# Autodesk Inventor assembly: Assembly1TankDrive
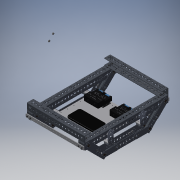
[picture p0: Inventor's stored thumbnail of the model, 180x180]
Saved by Autodesk Inventor 2016 (Build 200138000, 138)
## iProperties
Created: 2015-09-29
Part Number: Assembly1TankDrive
Document SubType Name: Assembly
Designer: phiro
Author: phiro
## Documents named in this file (15)
- C:\Users\phiro\Documents\GitHub\phi_robotics\3d-models\FTC_Tetrix_KOP_Block_Party\Troy designs\Assembly1TankDrive.iam
- C:\Users\phiro\Documents\GitHub\phi_robotics\3d-models\FTC_Tetrix_KOP_Block_Party\Tetrix_Kit_FTC\Autodesk Inventor Files\tetrix_c_channel-5.ipt
- C:\Users\phiro\Documents\GitHub\phi_robotics\3d-models\FTC_Tetrix_KOP_Block_Party\Tetrix_Kit_FTC\Autodesk Inventor Files\tetrix_739061_2012.ipt
- C:\Users\phiro\Documents\GitHub\phi_robotics\3d-models\FTC_Tetrix_KOP_Block_Party\Tetrix_Kit_FTC\Autodesk Inventor Files\tetrix_c_channel-2.ipt
- C:\Users\phiro\Documents\GitHub\phi_robotics\3d-models\FTC_Tetrix_KOP_Block_Party\Tetrix_Kit_FTC\Autodesk Inventor Files\tetrix_c_channel-3.ipt
- C:\Users\phiro\Documents\GitHub\phi_robotics\3d-models\FTC_Tetrix_KOP_Block_Party\Tetrix_Kit_FTC\Autodesk Inventor Files\tetrix_c_channel-4.ipt
- C:\Users\phiro\Documents\GitHub\phi_robotics\3d-models\FTC_Tetrix_KOP_Block_Party\Tetrix_Kit_FTC\Autodesk Inventor Files\tetrix_Lbracket-round.ipt
- C:\Users\phiro\Documents\GitHub\phi_robotics\3d-models\FTC_Tetrix_KOP_Block_Party\Tetrix_Kit_FTC\Autodesk Inventor Files\tetrix_flat_bar-288 MM.ipt
- C:\Users\phiro\Documents\GitHub\phi_robotics\3d-models\FTC_Tetrix_KOP_Block_Party\Tetrix_Kit_FTC\Autodesk Inventor Files\tetrix_screw-short.ipt
- C:\Users\phiro\Documents\GitHub\phi_robotics\3d-models\FTC_Tetrix_KOP_Block_Party\Tetrix_Kit_FTC\Autodesk Inventor Files\tetrix_lock_nut.ipt
- C:\Users\phiro\Documents\GitHub\phi_robotics\3d-models\FTC_Tetrix_KOP_Block_Party\Tetrix_Kit_FTC\Autodesk Inventor Files\tetrix_bushing.ipt
- C:\Users\phiro\Documents\GitHub\phi_robotics\3d-models\FTC_Tetrix_KOP_Block_Party\Tim Bloot Designs\MCPlate2.ipt
- C:\Users\phiro\Documents\GitHub\phi_robotics\3d-models\FTC_Tetrix_KOP_Block_Party\Tetrix_Kit_FTC\Autodesk Inventor Files\tetrix_739274_2013.ipt
- C:\Users\phiro\Documents\GitHub\phi_robotics\3d-models\FTC_Tetrix_KOP_Block_Party\Tim Bloot Designs\Andoid Phone.ipt
- C:\Users\phiro\Documents\GitHub\phi_robotics\3d-models\FTC_Tetrix_KOP_Block_Party\Tetrix_Kit_FTC\Autodesk Inventor Files\tetrix_motor_controller.ipt
## Components (222 placed, 14 different names)
1. tetrix_739061_2012:1 — Rigid:2, Rigid:58, Rigid:162, Rigid:163, Rigid:164, Rigid:165
2. tetrix_739061_2012:2 — Rigid:1, Rigid:3, Rigid:59, Rigid:166, Rigid:167, Rigid:168, Rigid:169
3. tetrix_c_channel-2:1 — Rigid:3, Rigid:6, Rigid:8, Rigid:196, Rigid:197, Rigid:198, Rigid:199, Rigid:212, Rigid:213, Rigid:214, Rigid:215
4. tetrix_739061_2012:3 — Rigid:4, Rigid:61, Rigid:178, Rigid:179, Rigid:180, Rigid:181
5. tetrix_739061_2012:4 — Rigid:5, Rotational:1, Rigid:60, Rigid:150, Rigid:151, Rigid:152, Rigid:153
6. tetrix_c_channel-2:2 — Rotational:1, Rigid:7, Rigid:9, Rigid:204, Rigid:205, Rigid:206, Rigid:207, Rigid:220, Rigid:221, Rigid:222, Rigid:223
7. tetrix_c_channel-3:1 — Rigid:10, Rigid:202, Rigid:203, Rigid:218, Rigid:219
8. tetrix_739061_2012:5 — Rigid:7, Rigid:10, Rigid:69, Rigid:174, Rigid:175, Rigid:176, Rigid:177
9. tetrix_739061_2012:6 — Rigid:9, Rigid:65, Rigid:154, Rigid:155, Rigid:156, Rigid:157
10. tetrix_739061_2012:7 — Rigid:8, Rigid:64, Rigid:158, Rigid:159, Rigid:160, Rigid:161
11. tetrix_739061_2012:8 — Rigid:6, Rigid:68, Rigid:170, Rigid:171, Rigid:172, Rigid:173
12. tetrix_c_channel-5:2 — Rigid:22, Rigid:23, Rigid:27, Rigid:29, Rigid:102, Rigid:103, Rigid:116, Rigid:117, Rigid:134, Rigid:135, Rigid:148, Rigid:149, Rigid:182, Rigid:183
13. tetrix_739061_2012:9 — Rigid:55, Rigid:86, Rigid:87, Rigid:88, Rigid:89
14. tetrix_739061_2012:10 — Rigid:54, Rigid:118, Rigid:119, Rigid:120, Rigid:121
15. tetrix_c_channel-2:3 — Rigid:104, Rigid:105, Rigid:106, Rigid:107, Rigid:136, Rigid:137, Rigid:138, Rigid:139
16. tetrix_739061_2012:11 — Rigid:56, Rigid:130, Rigid:131, Rigid:132, Rigid:133
17. tetrix_739061_2012:12 — Rotational:2, Rigid:57, Rigid:92, Rigid:93, Rigid:94, Rigid:95
18. tetrix_739061_2012:15 — Rigid:67, Rigid:90, Rigid:91, Rigid:100, Rigid:101
19. tetrix_739061_2012:16 — Rigid:62, Rigid:122, Rigid:123, Rigid:124, Rigid:125
20. tetrix_c_channel-4:1 — Rigid:21, Rigid:22, Rigid:70, Rigid:71, Rigid:74, Rigid:75
21. tetrix_c_channel-4:2 — Rigid:23, Rigid:72, Rigid:73, Rigid:76, Rigid:77
22. tetrix_c_channel-2:4 — Rotational:2, Rigid:24, Rigid:25, Rigid:112, Rigid:113, Rigid:114, Rigid:115, Rigid:144, Rigid:145, Rigid:146, Rigid:147
23. tetrix_739061_2012:17 — Rigid:24, Rigid:26, Rigid:63, Rigid:126, Rigid:127, Rigid:128, Rigid:129
24. tetrix_739061_2012:18 — Rigid:25, Rigid:66, Rigid:96, Rigid:97, Rigid:98, Rigid:99
25. tetrix_c_channel-3:2 — Rigid:26, Rigid:110, Rigid:111, Rigid:142, Rigid:143
26. tetrix_Lbracket-round:1 — Rigid:27, Rigid:31, Rigid:34, Rigid:36, Rigid:78, Rigid:79
27. tetrix_Lbracket-round:2 — Rigid:28, Rigid:39, Rigid:40, Rigid:82, Rigid:83
28. tetrix_Lbracket-round:3 — Rigid:29, Rigid:43, Rigid:44, Rigid:80, Rigid:81
29. tetrix_Lbracket-round:4 — Rigid:30, Rigid:32, Rigid:47, Rigid:48, Rigid:84, Rigid:85
30. tetrix_flat_bar-288 MM:1 — Rigid:31, Rigid:33, Rigid:35, Rigid:37, Rigid:38
31. tetrix_flat_bar-288 MM:2 — Rigid:32, Rigid:41, Rigid:42, Rigid:45, Rigid:46
32. tetrix_screw-short:1 — Rigid:33
33. tetrix_lock_nut:1 — Rigid:34
34. tetrix_screw-short:2 — Rigid:35
35. tetrix_screw-short:3 — Rigid:38
36. tetrix_screw-short:4 — Rigid:37
37. tetrix_screw-short:5 — Rigid:41
38. tetrix_screw-short:6 — Rigid:42
39. tetrix_screw-short:7 — Rigid:46
40. tetrix_screw-short:8 — Rigid:45
41. tetrix_lock_nut:2 — Rigid:36
42. tetrix_lock_nut:3 — Rigid:39
43. tetrix_lock_nut:4 — Rigid:40
44. tetrix_lock_nut:5 — Rigid:43
45. tetrix_lock_nut:6 — Rigid:44
46. tetrix_lock_nut:7 — Rigid:47
47. tetrix_lock_nut:8 — Rigid:48
48. tetrix_bushing:1 — Rigid:54
49. tetrix_bushing:2 — Rigid:56
50. tetrix_bushing:3 — Rigid:55
51. tetrix_bushing:4 — Rigid:57
52. tetrix_bushing:5 — Rigid:58
53. tetrix_bushing:6 — Rigid:60
54. tetrix_bushing:8 — Rigid:61
55. tetrix_bushing:9 — Rigid:59
56. tetrix_bushing:10 — Rigid:66
57. tetrix_bushing:11 — Rigid:67
58. tetrix_bushing:12 — Rigid:64
59. tetrix_bushing:13 — Rigid:65
60. tetrix_bushing:14 — Rigid:63
61. tetrix_bushing:15 — Rigid:62
62. tetrix_bushing:16 — Rigid:68
63. tetrix_bushing:17 — Rigid:69
64. tetrix_screw-short:9 — Rigid:71
65. tetrix_screw-short:10 — Rigid:70
66. tetrix_screw-short:11 — Rigid:72
67. tetrix_screw-short:12 — Rigid:73
68. tetrix_screw-short:13 — Rigid:77
69. tetrix_screw-short:14 — Rigid:76
70. tetrix_screw-short:15 — Rigid:75
71. tetrix_screw-short:16 — Rigid:74
72. tetrix_lock_nut:9 — Rigid:78
73. tetrix_lock_nut:10 — Rigid:79
74. tetrix_lock_nut:11 — Rigid:80
75. tetrix_lock_nut:12 — Rigid:81
76. tetrix_lock_nut:13 — Rigid:84
77. tetrix_lock_nut:14 — Rigid:85
78. tetrix_lock_nut:15 — Rigid:82
79. tetrix_lock_nut:16 — Rigid:83
80. tetrix_screw-short:17 — Rigid:87
81. tetrix_screw-short:18 — Rigid:86
82. tetrix_screw-short:19 — Rigid:91
83. tetrix_screw-short:20 — Rigid:89
84. tetrix_screw-short:21 — Rigid:90
85. tetrix_screw-short:22 — Rigid:88
86. tetrix_screw-short:23 — Rigid:95
87. tetrix_screw-short:24 — Rigid:94
88. tetrix_screw-short:25 — Rigid:97
89. tetrix_screw-short:26 — Rigid:96
90. tetrix_screw-short:27 — Rigid:93
91. tetrix_screw-short:28 — Rigid:92
92. tetrix_screw-short:29 — Rigid:99
93. tetrix_screw-short:30 — Rigid:98
94. tetrix_screw-short:31 — Rigid:100, Rigid:108
95. tetrix_screw-short:32 — Rigid:101, Rigid:109
96. tetrix_lock_nut:17 — Rigid:102
97. tetrix_lock_nut:18 — Rigid:103
98. tetrix_lock_nut:19 — Rigid:104
99. tetrix_lock_nut:20 — Rigid:105
100. tetrix_lock_nut:21 — Rigid:106
101. tetrix_lock_nut:22 — Rigid:107
102. tetrix_lock_nut:23 — Rigid:108
103. tetrix_lock_nut:24 — Rigid:109
104. tetrix_lock_nut:25 — Rigid:110
105. tetrix_lock_nut:26 — Rigid:111
106. tetrix_lock_nut:27 — Rigid:112
107. tetrix_lock_nut:28 — Rigid:113
108. tetrix_lock_nut:29 — Rigid:114
109. tetrix_lock_nut:30 — Rigid:115
110. tetrix_lock_nut:31 — Rigid:116
111. tetrix_lock_nut:32 — Rigid:117
112. tetrix_screw-short:33 — Rigid:119
113. tetrix_screw-short:34 — Rigid:118
114. tetrix_screw-short:35 — Rigid:120
115. tetrix_screw-short:36 — Rigid:121
116. tetrix_screw-short:37 — Rigid:122
117. tetrix_screw-short:38 — Rigid:123
118. tetrix_screw-short:39 — Rigid:124, Rigid:140
119. tetrix_screw-short:40 — Rigid:125, Rigid:141
120. tetrix_screw-short:41 — Rigid:126
121. tetrix_screw-short:42 — Rigid:127
122. tetrix_screw-short:43 — Rigid:128
123. tetrix_screw-short:44 — Rigid:129
124. tetrix_screw-short:45 — Rigid:130
125. tetrix_screw-short:46 — Rigid:131
126. tetrix_screw-short:47 — Rigid:132
127. tetrix_screw-short:48 — Rigid:133
128. tetrix_lock_nut:33 — Rigid:134
129. tetrix_lock_nut:34 — Rigid:135
130. tetrix_lock_nut:35 — Rigid:136
131. tetrix_lock_nut:36 — Rigid:137
132. tetrix_lock_nut:37 — Rigid:138
133. tetrix_lock_nut:38 — Rigid:139
134. tetrix_lock_nut:39 — Rigid:140
135. tetrix_lock_nut:40 — Rigid:141
136. tetrix_lock_nut:41 — Rigid:142
137. tetrix_lock_nut:42 — Rigid:143
138. tetrix_lock_nut:43 — Rigid:144
139. tetrix_lock_nut:44 — Rigid:145
140. tetrix_lock_nut:45 — Rigid:146
141. tetrix_lock_nut:46 — Rigid:147
142. tetrix_lock_nut:47 — Rigid:148
143. tetrix_lock_nut:48 — Rigid:149
144. tetrix_screw-short:49 — Rigid:150
145. tetrix_screw-short:50 — Rigid:151
146. tetrix_screw-short:51 — Rigid:152
147. tetrix_screw-short:52 — Rigid:153
148. tetrix_screw-short:53 — Rigid:154
149. tetrix_screw-short:54 — Rigid:155
150. tetrix_screw-short:55 — Rigid:156
151. tetrix_screw-short:56 — Rigid:157
152. tetrix_screw-short:57 — Rigid:158, Rigid:217
153. tetrix_screw-short:58 — Rigid:159, Rigid:216
154. tetrix_screw-short:59 — Rigid:160
155. tetrix_screw-short:60 — Rigid:161
156. tetrix_screw-short:61 — Rigid:162
157. tetrix_screw-short:62 — Rigid:163
158. tetrix_screw-short:63 — Rigid:164
159. tetrix_screw-short:64 — Rigid:165
160. tetrix_screw-short:65 — Rigid:181
161. tetrix_screw-short:66 — Rigid:180
162. tetrix_screw-short:67 — Rigid:179
163. tetrix_screw-short:68 — Rigid:178
164. tetrix_screw-short:69 — Rigid:177
165. tetrix_screw-short:70 — Rigid:176
166. tetrix_screw-short:71 — Rigid:175
167. tetrix_screw-short:72 — Rigid:174
168. tetrix_screw-short:73 — Rigid:173, Rigid:201
169. tetrix_screw-short:74 — Rigid:172, Rigid:200
170. tetrix_screw-short:75 — Rigid:171
171. tetrix_screw-short:76 — Rigid:170
172. tetrix_screw-short:77 — Rigid:169
173. tetrix_screw-short:78 — Rigid:168
174. tetrix_screw-short:79 — Rigid:167
175. tetrix_screw-short:80 — Rigid:166
176. MCPlate2:1 — Rigid:192, Mate:1, Rigid:193, Rotational:3
177. tetrix_flat_bar-288 MM:3 — Rigid:190
178. tetrix_flat_bar-288 MM:4 — Rigid:191, Rigid:192
179. tetrix_739274_2013:1 — Rigid:183, Rigid:187
180. tetrix_739274_2013:2 — Rigid:182, Rigid:186
181. tetrix_739274_2013:3 — Rigid:185, Rigid:189
182. tetrix_739274_2013:4 — Rigid:184, Rigid:188
183. tetrix_Lbracket-round:5 — Rigid:188, Rigid:190
184. tetrix_Lbracket-round:6 — Rigid:189
185. tetrix_Lbracket-round:7 — Rigid:186
186. tetrix_Lbracket-round:8 — Rigid:187, Rigid:191
187. Andoid Phone:1 — Mate:1
188. tetrix_motor_controller:1 — Rigid:193
189. tetrix_motor_controller:2 — Rotational:3
190. tetrix_lock_nut:49 — Rigid:210
191. tetrix_lock_nut:50 — Rigid:211
192. tetrix_lock_nut:51 — Rigid:212
193. tetrix_lock_nut:52 — Rigid:213
194. tetrix_lock_nut:53 — Rigid:214
195. tetrix_lock_nut:54 — Rigid:215
196. tetrix_lock_nut:55 — Rigid:216
197. tetrix_lock_nut:56 — Rigid:217
198. tetrix_lock_nut:57 — Rigid:218
199. tetrix_lock_nut:58 — Rigid:219
200. tetrix_lock_nut:59 — Rigid:220
201. tetrix_lock_nut:60 — Rigid:221
202. tetrix_lock_nut:61 — Rigid:222
203. tetrix_lock_nut:62 — Rigid:223
204. tetrix_lock_nut:63
205. tetrix_lock_nut:64
206. tetrix_lock_nut:65 — Rigid:194
207. tetrix_lock_nut:66 — Rigid:195
208. tetrix_lock_nut:67 — Rigid:196
209. tetrix_lock_nut:68 — Rigid:197
210. tetrix_lock_nut:69 — Rigid:198
211. tetrix_lock_nut:70 — Rigid:200
212. tetrix_lock_nut:71 — Rigid:199
213. tetrix_lock_nut:72 — Rigid:201
214. tetrix_lock_nut:73 — Rigid:202
215. tetrix_lock_nut:74 — Rigid:203
216. tetrix_lock_nut:75 — Rigid:204
217. tetrix_lock_nut:76 — Rigid:205
218. tetrix_lock_nut:77 — Rigid:206
219. tetrix_lock_nut:78 — Rigid:207
220. tetrix_lock_nut:79 — Rigid:208
221. tetrix_lock_nut:80 — Rigid:209
222. tetrix_c_channel-5:1 — Rigid:1, Rigid:2, Rigid:4, Rigid:5, Rigid:21, Rigid:28, Rigid:30, Rigid:184, Rigid:185, Rigid:194, Rigid:195, Rigid:208, Rigid:209, Rigid:210, Rigid:211
## Relationships (219: WeldJoint 215, RevoluteJoint 3, Mate 1)
- Rigid:1 [WeldJoint]: tetrix_739061_2012:2 ↔ tetrix_c_channel-5:1
- Rigid:2 [WeldJoint]: tetrix_739061_2012:1 ↔ tetrix_c_channel-5:1
- Rigid:3 [WeldJoint]: tetrix_739061_2012:2 ↔ tetrix_c_channel-2:1
- Rigid:4 [WeldJoint]: tetrix_739061_2012:3 ↔ tetrix_c_channel-5:1
- Rigid:5 [WeldJoint]: tetrix_739061_2012:4 ↔ tetrix_c_channel-5:1
- Rotational:1 [RevoluteJoint]: tetrix_739061_2012:4 ↔ tetrix_c_channel-2:2
- Rigid:6 [WeldJoint]: tetrix_c_channel-2:1 ↔ tetrix_739061_2012:8
- Rigid:7 [WeldJoint]: tetrix_c_channel-2:2 ↔ tetrix_739061_2012:5
- Rigid:8 [WeldJoint]: tetrix_c_channel-2:1 ↔ tetrix_739061_2012:7
- Rigid:9 [WeldJoint]: tetrix_c_channel-2:2 ↔ tetrix_739061_2012:6
- Rigid:10 [WeldJoint]: tetrix_c_channel-3:1 ↔ tetrix_739061_2012:5
- [WeldJoint]: tetrix_c_channel-5:2 ↔ tetrix_739061_2012:10
- [WeldJoint]: tetrix_c_channel-5:2 ↔ tetrix_739061_2012:9
- [WeldJoint]: tetrix_739061_2012:10 ↔ tetrix_c_channel-2:3
- [WeldJoint]: tetrix_c_channel-5:2 ↔ tetrix_739061_2012:11
- [WeldJoint]: tetrix_c_channel-5:2 ↔ tetrix_739061_2012:12
- [WeldJoint]: tetrix_c_channel-2:3 ↔ tetrix_739061_2012:16
- [WeldJoint]: tetrix_c_channel-2:3 ↔ tetrix_739061_2012:15
- Rigid:21 [WeldJoint]: tetrix_c_channel-4:1 ↔ tetrix_c_channel-5:1
- Rigid:22 [WeldJoint]: tetrix_c_channel-5:2 ↔ tetrix_c_channel-4:1
- Rigid:23 [WeldJoint]: tetrix_c_channel-5:2 ↔ tetrix_c_channel-4:2
- Rotational:2 [RevoluteJoint]: tetrix_739061_2012:12 ↔ tetrix_c_channel-2:4
- Rigid:24 [WeldJoint]: tetrix_c_channel-2:4 ↔ tetrix_739061_2012:17
- Rigid:25 [WeldJoint]: tetrix_c_channel-2:4 ↔ tetrix_739061_2012:18
- Rigid:26 [WeldJoint]: tetrix_739061_2012:17 ↔ tetrix_c_channel-3:2
- Rigid:27 [WeldJoint]: tetrix_c_channel-5:2 ↔ tetrix_Lbracket-round:1
- Rigid:28 [WeldJoint]: tetrix_Lbracket-round:2 ↔ tetrix_c_channel-5:1
- Rigid:29 [WeldJoint]: tetrix_c_channel-5:2 ↔ tetrix_Lbracket-round:3
- Rigid:30 [WeldJoint]: tetrix_Lbracket-round:4 ↔ tetrix_c_channel-5:1
- Rigid:31 [WeldJoint]: tetrix_Lbracket-round:1 ↔ tetrix_flat_bar-288 MM:1
- Rigid:32 [WeldJoint]: tetrix_Lbracket-round:4 ↔ tetrix_flat_bar-288 MM:2
- Rigid:33 [WeldJoint]: tetrix_flat_bar-288 MM:1 ↔ tetrix_screw-short:1
- Rigid:34 [WeldJoint]: tetrix_Lbracket-round:1 ↔ tetrix_lock_nut:1
- Rigid:35 [WeldJoint]: tetrix_flat_bar-288 MM:1 ↔ tetrix_screw-short:2
- Rigid:36 [WeldJoint]: tetrix_Lbracket-round:1 ↔ tetrix_lock_nut:2
- Rigid:37 [WeldJoint]: tetrix_flat_bar-288 MM:1 ↔ tetrix_screw-short:4
- Rigid:38 [WeldJoint]: tetrix_flat_bar-288 MM:1 ↔ tetrix_screw-short:3
- Rigid:39 [WeldJoint]: tetrix_Lbracket-round:2 ↔ tetrix_lock_nut:3
- Rigid:40 [WeldJoint]: tetrix_Lbracket-round:2 ↔ tetrix_lock_nut:4
- Rigid:41 [WeldJoint]: tetrix_flat_bar-288 MM:2 ↔ tetrix_screw-short:5
- Rigid:42 [WeldJoint]: tetrix_flat_bar-288 MM:2 ↔ tetrix_screw-short:6
- Rigid:43 [WeldJoint]: tetrix_Lbracket-round:3 ↔ tetrix_lock_nut:5
- Rigid:44 [WeldJoint]: tetrix_Lbracket-round:3 ↔ tetrix_lock_nut:6
- Rigid:45 [WeldJoint]: tetrix_flat_bar-288 MM:2 ↔ tetrix_screw-short:8
- Rigid:46 [WeldJoint]: tetrix_flat_bar-288 MM:2 ↔ tetrix_screw-short:7
- Rigid:47 [WeldJoint]: tetrix_Lbracket-round:4 ↔ tetrix_lock_nut:7
- Rigid:48 [WeldJoint]: tetrix_Lbracket-round:4 ↔ tetrix_lock_nut:8
- Rigid:54 [WeldJoint]: tetrix_739061_2012:10 ↔ tetrix_bushing:1
- Rigid:55 [WeldJoint]: tetrix_739061_2012:9 ↔ tetrix_bushing:3
- Rigid:56 [WeldJoint]: tetrix_739061_2012:11 ↔ tetrix_bushing:2
- Rigid:57 [WeldJoint]: tetrix_739061_2012:12 ↔ tetrix_bushing:4
- Rigid:58 [WeldJoint]: tetrix_739061_2012:1 ↔ tetrix_bushing:5
- Rigid:59 [WeldJoint]: tetrix_739061_2012:2 ↔ tetrix_bushing:9
- Rigid:60 [WeldJoint]: tetrix_739061_2012:4 ↔ tetrix_bushing:6
- Rigid:61 [WeldJoint]: tetrix_739061_2012:3 ↔ tetrix_bushing:8
- Rigid:62 [WeldJoint]: tetrix_739061_2012:16 ↔ tetrix_bushing:15
- Rigid:63 [WeldJoint]: tetrix_739061_2012:17 ↔ tetrix_bushing:14
- Rigid:64 [WeldJoint]: tetrix_739061_2012:7 ↔ tetrix_bushing:12
- Rigid:65 [WeldJoint]: tetrix_739061_2012:6 ↔ tetrix_bushing:13
- Rigid:66 [WeldJoint]: tetrix_739061_2012:18 ↔ tetrix_bushing:10
- Rigid:67 [WeldJoint]: tetrix_739061_2012:15 ↔ tetrix_bushing:11
- Rigid:68 [WeldJoint]: tetrix_739061_2012:8 ↔ tetrix_bushing:16
- Rigid:69 [WeldJoint]: tetrix_739061_2012:5 ↔ tetrix_bushing:17
- Rigid:70 [WeldJoint]: tetrix_c_channel-4:1 ↔ tetrix_screw-short:10
- Rigid:71 [WeldJoint]: tetrix_c_channel-4:1 ↔ tetrix_screw-short:9
- Rigid:72 [WeldJoint]: tetrix_c_channel-4:2 ↔ tetrix_screw-short:11
- Rigid:73 [WeldJoint]: tetrix_c_channel-4:2 ↔ tetrix_screw-short:12
- Rigid:74 [WeldJoint]: tetrix_c_channel-4:1 ↔ tetrix_screw-short:16
- Rigid:75 [WeldJoint]: tetrix_c_channel-4:1 ↔ tetrix_screw-short:15
- Rigid:76 [WeldJoint]: tetrix_c_channel-4:2 ↔ tetrix_screw-short:14
- Rigid:77 [WeldJoint]: tetrix_c_channel-4:2 ↔ tetrix_screw-short:13
- Rigid:78 [WeldJoint]: tetrix_Lbracket-round:1 ↔ tetrix_lock_nut:9
- Rigid:79 [WeldJoint]: tetrix_Lbracket-round:1 ↔ tetrix_lock_nut:10
- Rigid:80 [WeldJoint]: tetrix_Lbracket-round:3 ↔ tetrix_lock_nut:11
- Rigid:81 [WeldJoint]: tetrix_Lbracket-round:3 ↔ tetrix_lock_nut:12
- Rigid:82 [WeldJoint]: tetrix_Lbracket-round:2 ↔ tetrix_lock_nut:15
- Rigid:83 [WeldJoint]: tetrix_Lbracket-round:2 ↔ tetrix_lock_nut:16
- Rigid:84 [WeldJoint]: tetrix_Lbracket-round:4 ↔ tetrix_lock_nut:13
- Rigid:85 [WeldJoint]: tetrix_Lbracket-round:4 ↔ tetrix_lock_nut:14
- Rigid:86 [WeldJoint]: tetrix_739061_2012:9 ↔ tetrix_screw-short:18
- Rigid:87 [WeldJoint]: tetrix_739061_2012:9 ↔ tetrix_screw-short:17
- Rigid:88 [WeldJoint]: tetrix_739061_2012:9 ↔ tetrix_screw-short:22
- Rigid:89 [WeldJoint]: tetrix_739061_2012:9 ↔ tetrix_screw-short:20
- Rigid:90 [WeldJoint]: tetrix_739061_2012:15 ↔ tetrix_screw-short:21
- Rigid:91 [WeldJoint]: tetrix_739061_2012:15 ↔ tetrix_screw-short:19
- Rigid:92 [WeldJoint]: tetrix_739061_2012:12 ↔ tetrix_screw-short:28
- Rigid:93 [WeldJoint]: tetrix_739061_2012:12 ↔ tetrix_screw-short:27
- Rigid:94 [WeldJoint]: tetrix_739061_2012:12 ↔ tetrix_screw-short:24
- Rigid:95 [WeldJoint]: tetrix_739061_2012:12 ↔ tetrix_screw-short:23
- Rigid:96 [WeldJoint]: tetrix_739061_2012:18 ↔ tetrix_screw-short:26
- Rigid:97 [WeldJoint]: tetrix_739061_2012:18 ↔ tetrix_screw-short:25
- Rigid:98 [WeldJoint]: tetrix_739061_2012:18 ↔ tetrix_screw-short:30
- Rigid:99 [WeldJoint]: tetrix_739061_2012:18 ↔ tetrix_screw-short:29
- Rigid:100 [WeldJoint]: tetrix_739061_2012:15 ↔ tetrix_screw-short:31
- Rigid:101 [WeldJoint]: tetrix_739061_2012:15 ↔ tetrix_screw-short:32
- Rigid:102 [WeldJoint]: tetrix_c_channel-5:2 ↔ tetrix_lock_nut:17
- Rigid:103 [WeldJoint]: tetrix_c_channel-5:2 ↔ tetrix_lock_nut:18
- Rigid:104 [WeldJoint]: tetrix_c_channel-2:3 ↔ tetrix_lock_nut:19
- Rigid:105 [WeldJoint]: tetrix_c_channel-2:3 ↔ tetrix_lock_nut:20
- Rigid:106 [WeldJoint]: tetrix_c_channel-2:3 ↔ tetrix_lock_nut:21
- Rigid:107 [WeldJoint]: tetrix_c_channel-2:3 ↔ tetrix_lock_nut:22
- Rigid:108 [WeldJoint] (3 mm): tetrix_screw-short:31 ↔ tetrix_lock_nut:23
- Rigid:109 [WeldJoint] (3 mm): tetrix_screw-short:32 ↔ tetrix_lock_nut:24
- Rigid:110 [WeldJoint]: tetrix_c_channel-3:2 ↔ tetrix_lock_nut:25
- Rigid:111 [WeldJoint]: tetrix_c_channel-3:2 ↔ tetrix_lock_nut:26
- Rigid:112 [WeldJoint]: tetrix_c_channel-2:4 ↔ tetrix_lock_nut:27
- Rigid:113 [WeldJoint]: tetrix_c_channel-2:4 ↔ tetrix_lock_nut:28
- Rigid:114 [WeldJoint]: tetrix_c_channel-2:4 ↔ tetrix_lock_nut:29
- Rigid:115 [WeldJoint]: tetrix_c_channel-2:4 ↔ tetrix_lock_nut:30
- Rigid:116 [WeldJoint]: tetrix_c_channel-5:2 ↔ tetrix_lock_nut:31
- Rigid:117 [WeldJoint]: tetrix_c_channel-5:2 ↔ tetrix_lock_nut:32
- Rigid:118 [WeldJoint]: tetrix_739061_2012:10 ↔ tetrix_screw-short:34
- Rigid:119 [WeldJoint]: tetrix_739061_2012:10 ↔ tetrix_screw-short:33
- Rigid:120 [WeldJoint]: tetrix_739061_2012:10 ↔ tetrix_screw-short:35
- Rigid:121 [WeldJoint]: tetrix_739061_2012:10 ↔ tetrix_screw-short:36
- Rigid:122 [WeldJoint]: tetrix_739061_2012:16 ↔ tetrix_screw-short:37
- Rigid:123 [WeldJoint]: tetrix_739061_2012:16 ↔ tetrix_screw-short:38
- Rigid:124 [WeldJoint]: tetrix_739061_2012:16 ↔ tetrix_screw-short:39
- Rigid:125 [WeldJoint]: tetrix_739061_2012:16 ↔ tetrix_screw-short:40
- Rigid:126 [WeldJoint]: tetrix_739061_2012:17 ↔ tetrix_screw-short:41
- Rigid:127 [WeldJoint]: tetrix_739061_2012:17 ↔ tetrix_screw-short:42
- Rigid:128 [WeldJoint]: tetrix_739061_2012:17 ↔ tetrix_screw-short:43
- Rigid:129 [WeldJoint]: tetrix_739061_2012:17 ↔ tetrix_screw-short:44
- Rigid:130 [WeldJoint]: tetrix_739061_2012:11 ↔ tetrix_screw-short:45
- Rigid:131 [WeldJoint]: tetrix_739061_2012:11 ↔ tetrix_screw-short:46
- Rigid:132 [WeldJoint]: tetrix_739061_2012:11 ↔ tetrix_screw-short:47
- Rigid:133 [WeldJoint]: tetrix_739061_2012:11 ↔ tetrix_screw-short:48
- Rigid:134 [WeldJoint]: tetrix_c_channel-5:2 ↔ tetrix_lock_nut:33
- Rigid:135 [WeldJoint]: tetrix_c_channel-5:2 ↔ tetrix_lock_nut:34
- Rigid:136 [WeldJoint]: tetrix_c_channel-2:3 ↔ tetrix_lock_nut:35
- Rigid:137 [WeldJoint]: tetrix_c_channel-2:3 ↔ tetrix_lock_nut:36
- Rigid:138 [WeldJoint]: tetrix_c_channel-2:3 ↔ tetrix_lock_nut:37
- Rigid:139 [WeldJoint]: tetrix_c_channel-2:3 ↔ tetrix_lock_nut:38
- Rigid:140 [WeldJoint] (3 mm): tetrix_screw-short:39 ↔ tetrix_lock_nut:39
- Rigid:141 [WeldJoint] (3 mm): tetrix_screw-short:40 ↔ tetrix_lock_nut:40
- Rigid:142 [WeldJoint]: tetrix_c_channel-3:2 ↔ tetrix_lock_nut:41
- Rigid:143 [WeldJoint]: tetrix_c_channel-3:2 ↔ tetrix_lock_nut:42
- Rigid:144 [WeldJoint]: tetrix_c_channel-2:4 ↔ tetrix_lock_nut:43
- Rigid:145 [WeldJoint]: tetrix_c_channel-2:4 ↔ tetrix_lock_nut:44
- Rigid:146 [WeldJoint]: tetrix_c_channel-2:4 ↔ tetrix_lock_nut:45
- Rigid:147 [WeldJoint]: tetrix_c_channel-2:4 ↔ tetrix_lock_nut:46
- Rigid:148 [WeldJoint]: tetrix_c_channel-5:2 ↔ tetrix_lock_nut:47
- Rigid:149 [WeldJoint]: tetrix_c_channel-5:2 ↔ tetrix_lock_nut:48
- Rigid:150 [WeldJoint]: tetrix_739061_2012:4 ↔ tetrix_screw-short:49
- Rigid:151 [WeldJoint]: tetrix_739061_2012:4 ↔ tetrix_screw-short:50
- Rigid:152 [WeldJoint]: tetrix_739061_2012:4 ↔ tetrix_screw-short:51
- Rigid:153 [WeldJoint]: tetrix_739061_2012:4 ↔ tetrix_screw-short:52
- Rigid:154 [WeldJoint]: tetrix_739061_2012:6 ↔ tetrix_screw-short:53
- Rigid:155 [WeldJoint]: tetrix_739061_2012:6 ↔ tetrix_screw-short:54
- Rigid:156 [WeldJoint]: tetrix_739061_2012:6 ↔ tetrix_screw-short:55
- Rigid:157 [WeldJoint]: tetrix_739061_2012:6 ↔ tetrix_screw-short:56
- Rigid:158 [WeldJoint]: tetrix_739061_2012:7 ↔ tetrix_screw-short:57
- Rigid:159 [WeldJoint]: tetrix_739061_2012:7 ↔ tetrix_screw-short:58
- Rigid:160 [WeldJoint]: tetrix_739061_2012:7 ↔ tetrix_screw-short:59
- Rigid:161 [WeldJoint]: tetrix_739061_2012:7 ↔ tetrix_screw-short:60
- Rigid:162 [WeldJoint]: tetrix_739061_2012:1 ↔ tetrix_screw-short:61
- Rigid:163 [WeldJoint]: tetrix_739061_2012:1 ↔ tetrix_screw-short:62
- Rigid:164 [WeldJoint]: tetrix_739061_2012:1 ↔ tetrix_screw-short:63
- Rigid:165 [WeldJoint]: tetrix_739061_2012:1 ↔ tetrix_screw-short:64
- Rigid:166 [WeldJoint]: tetrix_739061_2012:2 ↔ tetrix_screw-short:80
- Rigid:167 [WeldJoint]: tetrix_739061_2012:2 ↔ tetrix_screw-short:79
- Rigid:168 [WeldJoint]: tetrix_739061_2012:2 ↔ tetrix_screw-short:78
- Rigid:169 [WeldJoint]: tetrix_739061_2012:2 ↔ tetrix_screw-short:77
- Rigid:170 [WeldJoint]: tetrix_739061_2012:8 ↔ tetrix_screw-short:76
- Rigid:171 [WeldJoint]: tetrix_739061_2012:8 ↔ tetrix_screw-short:75
- Rigid:172 [WeldJoint]: tetrix_739061_2012:8 ↔ tetrix_screw-short:74
- Rigid:173 [WeldJoint]: tetrix_739061_2012:8 ↔ tetrix_screw-short:73
- Rigid:174 [WeldJoint]: tetrix_739061_2012:5 ↔ tetrix_screw-short:72
- Rigid:175 [WeldJoint]: tetrix_739061_2012:5 ↔ tetrix_screw-short:71
- Rigid:176 [WeldJoint]: tetrix_739061_2012:5 ↔ tetrix_screw-short:70
- Rigid:177 [WeldJoint]: tetrix_739061_2012:5 ↔ tetrix_screw-short:69
- Rigid:178 [WeldJoint]: tetrix_739061_2012:3 ↔ tetrix_screw-short:68
- Rigid:179 [WeldJoint]: tetrix_739061_2012:3 ↔ tetrix_screw-short:67
- Rigid:180 [WeldJoint]: tetrix_739061_2012:3 ↔ tetrix_screw-short:66
- Rigid:181 [WeldJoint]: tetrix_739061_2012:3 ↔ tetrix_screw-short:65
- Rigid:182 [WeldJoint]: tetrix_c_channel-5:2 ↔ tetrix_739274_2013:2
- Rigid:183 [WeldJoint]: tetrix_c_channel-5:2 ↔ tetrix_739274_2013:1
- Rigid:184 [WeldJoint]: tetrix_739274_2013:4 ↔ tetrix_c_channel-5:1
- Rigid:185 [WeldJoint]: tetrix_739274_2013:3 ↔ tetrix_c_channel-5:1
- Rigid:186 [WeldJoint]: tetrix_739274_2013:2 ↔ tetrix_Lbracket-round:7
- Rigid:187 [WeldJoint]: tetrix_739274_2013:1 ↔ tetrix_Lbracket-round:8
- Rigid:188 [WeldJoint]: tetrix_739274_2013:4 ↔ tetrix_Lbracket-round:5
- Rigid:189 [WeldJoint]: tetrix_739274_2013:3 ↔ tetrix_Lbracket-round:6
- Rigid:190 [WeldJoint]: tetrix_flat_bar-288 MM:3 ↔ tetrix_Lbracket-round:5
- Rigid:191 [WeldJoint]: tetrix_flat_bar-288 MM:4 ↔ tetrix_Lbracket-round:8
- Rigid:192 [WeldJoint]: MCPlate2:1 ↔ tetrix_flat_bar-288 MM:4
- Mate:1: MCPlate2:1 ↔ Andoid Phone:1
- Rigid:193 [WeldJoint]: MCPlate2:1 ↔ tetrix_motor_controller:1
- Rotational:3 [RevoluteJoint]: MCPlate2:1 ↔ tetrix_motor_controller:2
- Rigid:194 [WeldJoint]: tetrix_lock_nut:65 ↔ tetrix_c_channel-5:1
- Rigid:195 [WeldJoint]: tetrix_lock_nut:66 ↔ tetrix_c_channel-5:1
- Rigid:196 [WeldJoint]: tetrix_c_channel-2:1 ↔ tetrix_lock_nut:67
- Rigid:197 [WeldJoint]: tetrix_c_channel-2:1 ↔ tetrix_lock_nut:68
- Rigid:198 [WeldJoint]: tetrix_c_channel-2:1 ↔ tetrix_lock_nut:69
- Rigid:199 [WeldJoint]: tetrix_c_channel-2:1 ↔ tetrix_lock_nut:71
- Rigid:200 [WeldJoint] (3 mm): tetrix_screw-short:74 ↔ tetrix_lock_nut:70
- Rigid:201 [WeldJoint] (3 mm): tetrix_screw-short:73 ↔ tetrix_lock_nut:72
- Rigid:202 [WeldJoint]: tetrix_c_channel-3:1 ↔ tetrix_lock_nut:73
- Rigid:203 [WeldJoint]: tetrix_c_channel-3:1 ↔ tetrix_lock_nut:74
- Rigid:204 [WeldJoint]: tetrix_c_channel-2:2 ↔ tetrix_lock_nut:75
- Rigid:205 [WeldJoint]: tetrix_c_channel-2:2 ↔ tetrix_lock_nut:76
- Rigid:206 [WeldJoint]: tetrix_c_channel-2:2 ↔ tetrix_lock_nut:77
- Rigid:207 [WeldJoint]: tetrix_c_channel-2:2 ↔ tetrix_lock_nut:78
- Rigid:208 [WeldJoint]: tetrix_lock_nut:79 ↔ tetrix_c_channel-5:1
- Rigid:209 [WeldJoint]: tetrix_lock_nut:80 ↔ tetrix_c_channel-5:1
- Rigid:210 [WeldJoint]: tetrix_lock_nut:49 ↔ tetrix_c_channel-5:1
- Rigid:211 [WeldJoint]: tetrix_lock_nut:50 ↔ tetrix_c_channel-5:1
- Rigid:212 [WeldJoint]: tetrix_c_channel-2:1 ↔ tetrix_lock_nut:51
- Rigid:213 [WeldJoint]: tetrix_c_channel-2:1 ↔ tetrix_lock_nut:52
- Rigid:214 [WeldJoint]: tetrix_c_channel-2:1 ↔ tetrix_lock_nut:53
- Rigid:215 [WeldJoint]: tetrix_c_channel-2:1 ↔ tetrix_lock_nut:54
- Rigid:216 [WeldJoint]: tetrix_screw-short:58 ↔ tetrix_lock_nut:55
- Rigid:217 [WeldJoint]: tetrix_screw-short:57 ↔ tetrix_lock_nut:56
- Rigid:218 [WeldJoint]: tetrix_c_channel-3:1 ↔ tetrix_lock_nut:57
- Rigid:219 [WeldJoint]: tetrix_c_channel-3:1 ↔ tetrix_lock_nut:58
- Rigid:220 [WeldJoint]: tetrix_c_channel-2:2 ↔ tetrix_lock_nut:59
- Rigid:221 [WeldJoint]: tetrix_c_channel-2:2 ↔ tetrix_lock_nut:60
- Rigid:222 [WeldJoint]: tetrix_c_channel-2:2 ↔ tetrix_lock_nut:61
- Rigid:223 [WeldJoint]: tetrix_c_channel-2:2 ↔ tetrix_lock_nut:62
## Named parameters: d12_d0 = 0 mm, d13_d1 = 0 mm, d14_d2 = 0 mm, d15_d3 = 0 mm, d16_d4 = 0 mm, d19_d7 = 0 mm, d21_d9 = 0 mm
